# Autodesk Inventor assembly: pulley .25 inch bore + wheel
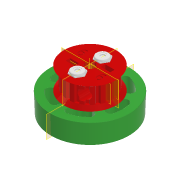
[picture p0: Inventor's stored thumbnail of the model, 180x180]
Saved by Autodesk Inventor 2020 (Build 240168000, 168)
## iProperties
Created: 2020-01-22
Part Number: pulley .25 inch bore + wheel
Document SubType Name: Assembly
Designer: ball
Author: ball
## Documents named in this file (6)
- C:\FTC\FTC8863CAD\2019 Robot\Collection\Intake\pulley .25 inch bore + wheel.iam
- C:\FTC\FTC8863CAD\2019 Robot\Generic Parts\18 tooth .2 pitch pulley 6mm D bore assembled from halves.iam
- C:\FTC\FTC8863CAD\Andymark\am-3572 2IN 8mm Compliant Wheel REV2.ipt
- C:\FTC\FTC8863CAD\StepLibraries\Nuts\6-32 NYLON-INSERT LOCKNUT.ipt
- C:\FTC\FTC8863CAD\StepLibraries\Washers\6 washer.ipt
- C:\FTC\FTC8863CAD\StepLibraries\Screws\6-32 x 1.125 SOCKET HEAD CAP SCREW.ipt
## Components (8 placed, 5 different names)
1. 18 tooth .2 pitch pulley 6mm D bore assembled from halves:1 [sub-assembly] — Mate:1, Mate:2, Flush:1, Mate:3, Mate:4, Angle:1, Mate:5, Mate:6, Angle:2
2. am-3572 2IN 8mm Compliant Wheel REV2:1 — Mate:1, Mate:2, Flush:1, Mate:7, Mate:8, Mate:9, Mate:10, Mate:13, Mate:14
3. 6-32 NYLON-INSERT LOCKNUT:1 — Mate:3, Mate:4, Angle:1
4. 6-32 NYLON-INSERT LOCKNUT:2 — Mate:5, Mate:6, Angle:2
5. 6 washer:1 — Mate:7, Mate:9, Mate:11
6. 6 washer:2 — Mate:8, Mate:10, Mate:12
7. 6-32 x 1.125 SOCKET HEAD CAP SCREW:1 — Mate:11, Mate:13
8. 6-32 x 1.125 SOCKET HEAD CAP SCREW:2 — Mate:12, Mate:14
## Relationships (17: Mate 14, Angle 2, Flush 1)
- Mate:1: 18 tooth .2 pitch pulley 6mm D bore assembled from halves:1 ↔ am-3572 2IN 8mm Compliant Wheel REV2:1
- Mate:2: 18 tooth .2 pitch pulley 6mm D bore assembled from halves:1 ↔ am-3572 2IN 8mm Compliant Wheel REV2:1
- Flush:1: 18 tooth .2 pitch pulley 6mm D bore assembled from halves:1 ↔ am-3572 2IN 8mm Compliant Wheel REV2:1
- Mate:3: 18 tooth .2 pitch pulley 6mm D bore assembled from halves:1 ↔ 6-32 NYLON-INSERT LOCKNUT:1
- Mate:4: 18 tooth .2 pitch pulley 6mm D bore assembled from halves:1 ↔ 6-32 NYLON-INSERT LOCKNUT:1
- Angle:1 (0 deg): 18 tooth .2 pitch pulley 6mm D bore assembled from halves:1 ↔ 6-32 NYLON-INSERT LOCKNUT:1
- Mate:5: 18 tooth .2 pitch pulley 6mm D bore assembled from halves:1 ↔ 6-32 NYLON-INSERT LOCKNUT:2
- Mate:6: 18 tooth .2 pitch pulley 6mm D bore assembled from halves:1 ↔ 6-32 NYLON-INSERT LOCKNUT:2
- Angle:2 (0 deg): 18 tooth .2 pitch pulley 6mm D bore assembled from halves:1 ↔ 6-32 NYLON-INSERT LOCKNUT:2
- Mate:7: am-3572 2IN 8mm Compliant Wheel REV2:1 ↔ 6 washer:1
- Mate:8: am-3572 2IN 8mm Compliant Wheel REV2:1 ↔ 6 washer:2
- Mate:9: am-3572 2IN 8mm Compliant Wheel REV2:1 ↔ 6 washer:1
- Mate:10: am-3572 2IN 8mm Compliant Wheel REV2:1 ↔ 6 washer:2
- Mate:11: 6 washer:1 ↔ 6-32 x 1.125 SOCKET HEAD CAP SCREW:1
- Mate:12: 6 washer:2 ↔ 6-32 x 1.125 SOCKET HEAD CAP SCREW:2
- Mate:13: am-3572 2IN 8mm Compliant Wheel REV2:1 ↔ 6-32 x 1.125 SOCKET HEAD CAP SCREW:1
- Mate:14: am-3572 2IN 8mm Compliant Wheel REV2:1 ↔ 6-32 x 1.125 SOCKET HEAD CAP SCREW:2
